# Autodesk Inventor assembly: Übung KO2 2023
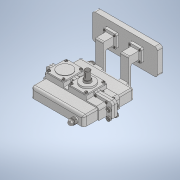
[picture p0: Inventor's stored thumbnail of the model, 180x180]
Saved by Autodesk Inventor 2022 (Build 260153000, 153)
## iProperties
Created: 2023-01-26
Part Number: Übung KO2 2023
Document SubType Name: Assembly
Designer: Matias Nicky
Author: Matias Nicky
## Documents named in this file (26)
- C:\Users\Matias Nicky\Documents\Nicky\HTW Fahrzeugtechnik\Semester 4\Konstruktion 2\Inventor\Übung KO2 2023.iam
- C:\Users\Matias Nicky\Documents\Nicky\HTW Fahrzeugtechnik\Semester 4\Konstruktion 2\Inventor\AbtriebswelleZahnrad 2.ipt
- C:\Users\Matias Nicky\Documents\Nicky\HTW Fahrzeugtechnik\Semester 4\Konstruktion 2\Inventor\AntriebswelleZahnrad 1.ipt
- C:\Users\Matias Nicky\Documents\Nicky\HTW Fahrzeugtechnik\Semester 4\Konstruktion 2\Inventor\Zahnrad2Rad2.ipt
- C:\Users\Matias Nicky\Documents\Inventor\Content Center Files\R2022\de-DE\DIN 471(2)\DIN 471 - 30 x 1,5(1).ipt
- C:\Users\Matias Nicky\Documents\Inventor\Content Center Files\R2022\de-DE\DIN 471(2)\DIN 471 - 35 x 1,5(1).ipt
- C:\Users\Matias Nicky\Documents\Inventor\Content Center Files\R2022\de-DE\DIN BEARING(1)\DIN 625 SKF - SKF 6006.ipt
- C:\Users\Matias Nicky\Documents\Nicky\HTW Fahrzeugtechnik\Semester 4\Konstruktion 2\Inventor\Gehäuse.ipt
- C:\Users\Matias Nicky\Documents\Nicky\HTW Fahrzeugtechnik\Semester 4\Konstruktion 2\Inventor\Gehäuse oben.ipt
- C:\Users\Matias Nicky\Documents\Inventor\Content Center Files\R2022\de-DE\DIN 3771(00)\DIN 3771 - 60 x 3,55 - N - NBR 70(1).ipt
- C:\Users\Matias Nicky\Documents\Inventor\Content Center Files\R2022\de-DE\DIN 6912\DIN 6912 - M10 x 30.ipt
- C:\Users\Matias Nicky\Documents\Inventor\Content Center Files\R2022\de-DE\ISO 4032(1)\ISO 4032 - M10DIN EN.ipt
- C:\Users\Matias Nicky\Documents\Inventor\Content Center Files\R2022\de-DE\DIN 6912\DIN 6912 - M6 x 30.ipt
- C:\Users\Matias Nicky\Documents\Inventor\Content Center Files\R2022\de-DE\DIN 6912\DIN 6912 - M5 x 30.ipt
- C:\Users\Matias Nicky\Documents\Inventor\Content Center Files\R2022\de-DE\ISO 4032(1)\ISO 4032 - M6DIN EN.ipt
- C:\Users\Matias Nicky\Documents\Inventor\Content Center Files\R2022\de-DE\ISO 4032(1)\ISO 4032 - M5DIN EN.ipt
- C:\Users\Matias Nicky\Documents\Nicky\HTW Fahrzeugtechnik\Semester 4\Konstruktion 2\Inventor\Deckel Endewelle.ipt
- C:\Users\Matias Nicky\Documents\Inventor\Content Center Files\R2022\de-DE\IS 7483\IS 7483 - M5 x 10.ipt
- C:\Users\Matias Nicky\Documents\Nicky\HTW Fahrzeugtechnik\Semester 4\Konstruktion 2\Inventor\Deckel verbindungswelle.ipt
- C:\Users\Matias Nicky\Documents\Inventor\Content Center Files\R2022\de-DE\ISO 6194_1(2)\ISO 6194_1 - 25x47x7-Typ 2.ipt
- C:\Users\Matias Nicky\Documents\Inventor\Content Center Files\R2022\de-DE\DIN 1587\DIN 1587 - M14 x 2.ipt
- C:\Users\Matias Nicky\Documents\Nicky\HTW Fahrzeugtechnik\Semester 4\Konstruktion 2\Inventor\Schmierung.ipt
- C:\Users\Matias Nicky\Documents\Inventor\Content Center Files\R2022\de-DE\DIN 6885-1 A\DIN 6885 - A 10 x 8 x 22.ipt
- C:\Users\Matias Nicky\Documents\Nicky\HTW Fahrzeugtechnik\Semester 4\Konstruktion 2\Inventor\Platte für Gehäuse.ipt
- C:\Users\Matias Nicky\Documents\Inventor\Content Center Files\R2022\de-DE\DIN 920\DIN 920 - M5 x 16.ipt
- C:\Users\Matias Nicky\Documents\Nicky\HTW Fahrzeugtechnik\Semester 4\Konstruktion 2\Inventor\Gehäuse festigung platte.ipt
## Components (94 placed, 25 different names)
1. AbtriebswelleZahnrad 2:1 — Passend:21, Passend:22, Passend:23, Passend:24, Passend:29, Passend:30, Passend:35, Fluchtend:1, Passend:38, Passend:40, Passend:47, Passend:98, Passend:102, Passend:126, Passend:129, Passend:133, Passend:134, Passend:135
2. AntriebswelleZahnrad 1:1 — Passend:17, Passend:25, Passend:26, Passend:27, Passend:28, Passend:35, Fluchtend:1, Passend:37, Passend:46, Passend:99, Passend:101, Passend:127, Passend:164
3. Zahnrad2Rad2:1 — Passend:126, Passend:129
4. DIN 471 > 9mm <= 300mm 30 x 1,5:2 — Passend:21, Passend:22, Passend:39
5. DIN 471 > 9mm <= 300mm 30 x 1,5:5 — Passend:23, Passend:24, Passend:43
6. DIN 471 > 9mm <= 300mm 35 x 1,5:1 — Passend:29, Passend:30
7. DIN 471 > 9mm <= 300mm 30 x 1,5:3 — Passend:17, Passend:25, Passend:26, Passend:44
8. DIN 471 > 9mm <= 300mm 30 x 1,5:4 — Passend:27, Passend:28, Passend:128
9. DIN 625 SKF SKF 6006:1 — Passend:19, Passend:38, Passend:43
10. DIN 625 SKF SKF 6006:2 — Passend:20, Passend:39, Passend:41, Passend:45
11. DIN 625 SKF SKF 6006:3 — Passend:32, Passend:37, Passend:42, Passend:127, Passend:128
12. DIN 625 SKF SKF 6006:4 — Passend:31, Passend:44
13. Gehäuse:1 — Passend:18, Passend:19, Passend:20, Passend:31, Passend:32, Passend:41, Passend:42, Passend:61, Passend:63, Passend:65, Passend:67, Passend:73, Passend:75, Passend:77, Passend:79, Passend:81, Passend:83, Einfügen:17, Einfügen:18, Passend:84, Fluchtend:6, Passend:85, Passend:86, Fluchtend:7, Passend:87, Passend:96, Passend:97, Passend:100, Passend:103, Passend:104, Passend:105, Passend:124, Passend:125, Fluchtend:8, Passend:130, Passend:131, Passend:132, Passend:136, Passend:137, Passend:138, Passend:139, Passend:140, Passend:141
14. Gehäuse oben:1 — Passend:18, Passend:40, Passend:45, Fluchtend:3, Fluchtend:5, Passend:50, Passend:51, Passend:52, Passend:53, Passend:56, Passend:57, Passend:58, Passend:59, Einfügen:9, Einfügen:10, Einfügen:11, Einfügen:12, Einfügen:13, Einfügen:14, Einfügen:15, Einfügen:16, Passend:122, Passend:123
15. DIN 3771 60 x 3,55 - N - NBR 70:1 — Passend:47, Fluchtend:2
16. DIN 3771 60 x 3,55 - N - NBR 70:2 — Passend:46, Fluchtend:4
17. DIN 6912 M10 x 30:5 — Passend:50, Passend:51, Passend:66
18. DIN 6912 M10 x 30:3 — Passend:52, Passend:53, Passend:60
19. DIN 6912 M10 x 30:2 — Passend:56, Passend:57, Passend:62
20. DIN 6912 M10 x 30:6 — Passend:58, Passend:59, Passend:64
21. DIN EN 24032 M10:1 — Passend:60, Passend:61
22. DIN EN 24032 M10:2 — Passend:62, Passend:63
23. DIN EN 24032 M10:3 — Passend:64, Passend:65
24. DIN EN 24032 M10:4 — Passend:66, Passend:67
25. DIN 6912 M5 x 30:1 — Einfügen:9, Passend:82
26. DIN 6912 M5 x 30:2 — Einfügen:10, Passend:80
27. DIN 6912 M5 x 30:3 — Einfügen:11, Passend:76
28. DIN 6912 M5 x 30:4 — Einfügen:12, Passend:72
29. DIN 6912 M5 x 30:5 — Einfügen:13, Passend:74
30. DIN 6912 M5 x 30:6 — Einfügen:14, Passend:78
31. DIN EN 24032 M5:1 — Passend:72, Passend:73
32. DIN EN 24032 M5:2 — Passend:74, Passend:75
33. DIN EN 24032 M5:3 — Passend:76, Passend:77
34. DIN EN 24032 M5:4 — Passend:78, Passend:79
35. DIN EN 24032 M5:5 — Passend:80, Passend:81
36. DIN EN 24032 M5:6 — Passend:82, Passend:83
37. DIN 6912 M6 x 30:1 — Einfügen:15
38. DIN 6912 M6 x 30:2 — Einfügen:16
39. DIN EN 24032 M6:1 — Einfügen:17
40. DIN EN 24032 M6:2 — Einfügen:18
41. Deckel Endewelle:1 — Passend:84, Fluchtend:6, Passend:85, Passend:88, Passend:89, Passend:90, Passend:91, Passend:92, Passend:93, Passend:94, Passend:95
42. Deckel Endewelle:2 — Passend:86, Fluchtend:7, Passend:87, Einfügen:19, Einfügen:20, Einfügen:21, Einfügen:22
43. IS 7483 M5 x 10:1 — Passend:88, Passend:89
44. IS 7483 M5 x 10:2 — Passend:90, Passend:91
45. IS 7483 M5 x 10:3 — Passend:92, Passend:93
46. IS 7483 M5 x 10:4 — Passend:94, Passend:95
47. IS 7483 M5 x 10:5 — Einfügen:19
48. IS 7483 M5 x 10:6 — Einfügen:20
49. IS 7483 M5 x 10:7 — Einfügen:21
50. IS 7483 M5 x 10:8 — Einfügen:22
51. Deckel verbindungswelle:1 — Passend:96, Passend:97, Passend:103, Passend:114, Passend:115, Passend:116, Passend:117, Passend:118, Passend:119, Passend:120, Passend:121
52. Deckel verbindungswelle:2 — Passend:100, Passend:104, Passend:105, Passend:106, Passend:107, Passend:108, Passend:109, Passend:110, Passend:111, Passend:112, Passend:113
53. ISO 6194/1 25x47x7-Typ 2:1 — Passend:98, Passend:102
54. ISO 6194/1 25x47x7-Typ 2:2 — Passend:99, Passend:101
55. IS 7483 M5 x 10:9 — Passend:106, Passend:107
56. IS 7483 M5 x 10:10 — Passend:108, Passend:109
57. IS 7483 M5 x 10:11 — Passend:110, Passend:111
58. IS 7483 M5 x 10:12 — Passend:112, Passend:113
59. IS 7483 M5 x 10:13 — Passend:114, Passend:115
60. IS 7483 M5 x 10:14 — Passend:116, Passend:117
61. IS 7483 M5 x 10:15 — Passend:118, Passend:119
62. IS 7483 M5 x 10:16 — Passend:120, Passend:121
63. DIN 1587 M14 - SW21:1 — Passend:122, Passend:123
64. DIN 1587 M14 - SW21:2 — Passend:124, Passend:125
65. Schmierung:1 — Passend:130, Passend:131, Passend:132
66. DIN 6885-1 A A 10 x 8 x 22:1 — Passend:133, Passend:134, Passend:135
67. Platte für Gehäuse:1 — Passend:139, Passend:140, Passend:141, Einfügen:23, Einfügen:24, Einfügen:25, Einfügen:26, Passend:142, Passend:143, Passend:144, Passend:146, Passend:148, Passend:149, Passend:150, Passend:151, Passend:152, Passend:153, Passend:154, Passend:155, Passend:156, Passend:157, Passend:158, Passend:159, Passend:160, Passend:161, Passend:162, Passend:163
68. Platte für Gehäuse:2 — Passend:136, Passend:137, Passend:138, Einfügen:27, Einfügen:28, Einfügen:29, Einfügen:30, Passend:145, Passend:147, Einfügen:31, Einfügen:32, Einfügen:33, Einfügen:34, Einfügen:35, Einfügen:36, Einfügen:37, Einfügen:38
69. DIN 920 M5 x 16:1 — Einfügen:23
70. DIN 920 M5 x 16:2 — Einfügen:24
71. DIN 920 M5 x 16:3 — Einfügen:25
72. DIN 920 M5 x 16:4 — Einfügen:26
73. DIN 920 M5 x 16:5 — Einfügen:27
74. DIN 920 M5 x 16:6 — Einfügen:28
75. DIN 920 M5 x 16:7 — Einfügen:29
76. DIN 920 M5 x 16:8 — Einfügen:30
77. Gehäuse festigung platte:1 — Passend:142, Passend:143, Passend:144
78. Gehäuse festigung platte:2 — Passend:145, Passend:146, Passend:147
79. DIN 920 M5 x 16:9 — Passend:148, Passend:149
80. DIN 920 M5 x 16:10 — Passend:150, Passend:151
81. DIN 920 M5 x 16:11 — Passend:152, Passend:153
82. DIN 920 M5 x 16:12 — Passend:154, Passend:155
83. DIN 920 M5 x 16:13 — Passend:156, Passend:157
84. DIN 920 M5 x 16:14 — Passend:158, Passend:159
85. DIN 920 M5 x 16:15 — Passend:160, Passend:161
86. DIN 920 M5 x 16:16 — Passend:162, Passend:163
87. DIN 920 M5 x 16:17 — Einfügen:31
88. DIN 920 M5 x 16:18 — Einfügen:32
89. DIN 920 M5 x 16:19 — Einfügen:33
90. DIN 920 M5 x 16:20 — Einfügen:34
91. DIN 920 M5 x 16:21 — Einfügen:35
92. DIN 920 M5 x 16:22 — Einfügen:36
93. DIN 920 M5 x 16:23 — Einfügen:37
94. DIN 920 M5 x 16:24 — Einfügen:38
## Relationships (175: Mate 137, Insert 30, Flush 8)
- Passend:17 [Mate]: AntriebswelleZahnrad 1:1 ↔ DIN 471 > 9mm <= 300mm 30 x 1,5:3
- Passend:18 [Mate]: Gehäuse:1 ↔ Gehäuse oben:1
- Passend:19 [Mate]: DIN 625 SKF SKF 6006:1 ↔ Gehäuse:1
- Passend:20 [Mate]: DIN 625 SKF SKF 6006:2 ↔ Gehäuse:1
- Passend:21 [Mate]: AbtriebswelleZahnrad 2:1 ↔ DIN 471 > 9mm <= 300mm 30 x 1,5:2
- Passend:22 [Mate]: AbtriebswelleZahnrad 2:1 ↔ DIN 471 > 9mm <= 300mm 30 x 1,5:2
- Passend:23 [Mate]: AbtriebswelleZahnrad 2:1 ↔ DIN 471 > 9mm <= 300mm 30 x 1,5:5
- Passend:24 [Mate]: AbtriebswelleZahnrad 2:1 ↔ DIN 471 > 9mm <= 300mm 30 x 1,5:5
- Passend:25 [Mate]: AntriebswelleZahnrad 1:1 ↔ DIN 471 > 9mm <= 300mm 30 x 1,5:3
- Passend:26 [Mate]: AntriebswelleZahnrad 1:1 ↔ DIN 471 > 9mm <= 300mm 30 x 1,5:3
- Passend:27 [Mate]: AntriebswelleZahnrad 1:1 ↔ DIN 471 > 9mm <= 300mm 30 x 1,5:4
- Passend:28 [Mate]: AntriebswelleZahnrad 1:1 ↔ DIN 471 > 9mm <= 300mm 30 x 1,5:4
- Passend:29 [Mate]: AbtriebswelleZahnrad 2:1 ↔ DIN 471 > 9mm <= 300mm 35 x 1,5:1
- Passend:30 [Mate]: AbtriebswelleZahnrad 2:1 ↔ DIN 471 > 9mm <= 300mm 35 x 1,5:1
- Passend:31 [Mate]: DIN 625 SKF SKF 6006:4 ↔ Gehäuse:1
- Passend:32 [Mate]: DIN 625 SKF SKF 6006:3 ↔ Gehäuse:1
- Passend:35 [Mate] (87 mm): AbtriebswelleZahnrad 2:1 ↔ AntriebswelleZahnrad 1:1
- Fluchtend:1 [Flush]: AbtriebswelleZahnrad 2:1 ↔ AntriebswelleZahnrad 1:1
- Passend:37 [Mate]: AntriebswelleZahnrad 1:1 ↔ DIN 625 SKF SKF 6006:3
- Passend:38 [Mate]: AbtriebswelleZahnrad 2:1 ↔ DIN 625 SKF SKF 6006:1
- Passend:39 [Mate]: DIN 471 > 9mm <= 300mm 30 x 1,5:2 ↔ DIN 625 SKF SKF 6006:2
- Passend:40 [Mate]: AbtriebswelleZahnrad 2:1 ↔ Gehäuse oben:1
- Passend:41 [Mate]: DIN 625 SKF SKF 6006:2 ↔ Gehäuse:1
- Passend:42 [Mate]: DIN 625 SKF SKF 6006:3 ↔ Gehäuse:1
- Passend:43 [Mate]: DIN 471 > 9mm <= 300mm 30 x 1,5:5 ↔ DIN 625 SKF SKF 6006:1
- Passend:44 [Mate]: DIN 471 > 9mm <= 300mm 30 x 1,5:3 ↔ DIN 625 SKF SKF 6006:4
- Passend:45 [Mate]: DIN 625 SKF SKF 6006:2 ↔ Gehäuse oben:1
- Passend:46 [Mate]: AntriebswelleZahnrad 1:1 ↔ DIN 3771 60 x 3,55 - N - NBR 70:2
- Passend:47 [Mate]: AbtriebswelleZahnrad 2:1 ↔ DIN 3771 60 x 3,55 - N - NBR 70:1
- Fluchtend:2 [Flush] (-1.775 mm): DIN 3771 60 x 3,55 - N - NBR 70:1
- Fluchtend:3 [Flush]: Gehäuse oben:1
- Fluchtend:4 [Flush] (-1.755 mm): DIN 3771 60 x 3,55 - N - NBR 70:2
- Fluchtend:5 [Flush]: Gehäuse oben:1
- Passend:50 [Mate]: Gehäuse oben:1 ↔ DIN 6912 M10 x 30:5
- Passend:51 [Mate]: Gehäuse oben:1 ↔ DIN 6912 M10 x 30:5
- Passend:52 [Mate]: Gehäuse oben:1 ↔ DIN 6912 M10 x 30:3
- Passend:53 [Mate]: Gehäuse oben:1 ↔ DIN 6912 M10 x 30:3
- Passend:56 [Mate]: Gehäuse oben:1 ↔ DIN 6912 M10 x 30:2
- Passend:57 [Mate]: Gehäuse oben:1 ↔ DIN 6912 M10 x 30:2
- Passend:58 [Mate]: Gehäuse oben:1 ↔ DIN 6912 M10 x 30:6
- Passend:59 [Mate]: Gehäuse oben:1 ↔ DIN 6912 M10 x 30:6
- Passend:60 [Mate]: DIN 6912 M10 x 30:3 ↔ DIN EN 24032 M10:1
- Passend:61 [Mate]: Gehäuse:1 ↔ DIN EN 24032 M10:1
- Passend:62 [Mate]: DIN 6912 M10 x 30:2 ↔ DIN EN 24032 M10:2
- Passend:63 [Mate]: Gehäuse:1 ↔ DIN EN 24032 M10:2
- Passend:64 [Mate]: DIN 6912 M10 x 30:6 ↔ DIN EN 24032 M10:3
- Passend:65 [Mate]: Gehäuse:1 ↔ DIN EN 24032 M10:3
- Passend:66 [Mate]: DIN 6912 M10 x 30:5 ↔ DIN EN 24032 M10:4
- Passend:67 [Mate]: Gehäuse:1 ↔ DIN EN 24032 M10:4
- Einfügen:9 [Insert]: Gehäuse oben:1 ↔ DIN 6912 M5 x 30:1
- Einfügen:10 [Insert]: Gehäuse oben:1 ↔ DIN 6912 M5 x 30:2
- Einfügen:11 [Insert]: Gehäuse oben:1 ↔ DIN 6912 M5 x 30:3
- Einfügen:12 [Insert]: Gehäuse oben:1 ↔ DIN 6912 M5 x 30:4
- Einfügen:13 [Insert]: Gehäuse oben:1 ↔ DIN 6912 M5 x 30:5
- Einfügen:14 [Insert]: Gehäuse oben:1 ↔ DIN 6912 M5 x 30:6
- Passend:72 [Mate]: DIN 6912 M5 x 30:4 ↔ DIN EN 24032 M5:1
- Passend:73 [Mate]: Gehäuse:1 ↔ DIN EN 24032 M5:1
- Passend:74 [Mate]: DIN 6912 M5 x 30:5 ↔ DIN EN 24032 M5:2
- Passend:75 [Mate]: Gehäuse:1 ↔ DIN EN 24032 M5:2
- Passend:76 [Mate]: DIN 6912 M5 x 30:3 ↔ DIN EN 24032 M5:3
- Passend:77 [Mate]: Gehäuse:1 ↔ DIN EN 24032 M5:3
- Passend:78 [Mate]: DIN 6912 M5 x 30:6 ↔ DIN EN 24032 M5:4
- Passend:79 [Mate]: Gehäuse:1 ↔ DIN EN 24032 M5:4
- Passend:80 [Mate]: DIN 6912 M5 x 30:2 ↔ DIN EN 24032 M5:5
- Passend:81 [Mate]: Gehäuse:1 ↔ DIN EN 24032 M5:5
- Passend:82 [Mate]: DIN 6912 M5 x 30:1 ↔ DIN EN 24032 M5:6
- Passend:83 [Mate]: Gehäuse:1 ↔ DIN EN 24032 M5:6
- Einfügen:15 [Insert]: Gehäuse oben:1 ↔ DIN 6912 M6 x 30:1
- Einfügen:16 [Insert]: Gehäuse oben:1 ↔ DIN 6912 M6 x 30:2
- Einfügen:17 [Insert]: Gehäuse:1 ↔ DIN EN 24032 M6:1
- Einfügen:18 [Insert]: Gehäuse:1 ↔ DIN EN 24032 M6:2
- Passend:84 [Mate]: Gehäuse:1 ↔ Deckel Endewelle:1
- Fluchtend:6 [Flush]: Gehäuse:1 ↔ Deckel Endewelle:1
- Passend:85 [Mate]: Gehäuse:1 ↔ Deckel Endewelle:1
- Passend:86 [Mate]: Gehäuse:1 ↔ Deckel Endewelle:2
- Fluchtend:7 [Flush]: Gehäuse:1 ↔ Deckel Endewelle:2
- Passend:87 [Mate]: Gehäuse:1 ↔ Deckel Endewelle:2
- Passend:88 [Mate]: Deckel Endewelle:1 ↔ IS 7483 M5 x 10:1
- Passend:89 [Mate]: Deckel Endewelle:1 ↔ IS 7483 M5 x 10:1
- Passend:90 [Mate]: Deckel Endewelle:1 ↔ IS 7483 M5 x 10:2
- Passend:91 [Mate]: Deckel Endewelle:1 ↔ IS 7483 M5 x 10:2
- Passend:92 [Mate]: Deckel Endewelle:1 ↔ IS 7483 M5 x 10:3
- Passend:93 [Mate]: Deckel Endewelle:1 ↔ IS 7483 M5 x 10:3
- Passend:94 [Mate]: Deckel Endewelle:1 ↔ IS 7483 M5 x 10:4
- Passend:95 [Mate]: Deckel Endewelle:1 ↔ IS 7483 M5 x 10:4
- Einfügen:19 [Insert]: Deckel Endewelle:2 ↔ IS 7483 M5 x 10:5
- Einfügen:20 [Insert]: Deckel Endewelle:2 ↔ IS 7483 M5 x 10:6
- Einfügen:21 [Insert]: Deckel Endewelle:2 ↔ IS 7483 M5 x 10:7
- Einfügen:22 [Insert]: Deckel Endewelle:2 ↔ IS 7483 M5 x 10:8
- Passend:96 [Mate]: Gehäuse:1 ↔ Deckel verbindungswelle:1
- Passend:97 [Mate]: Gehäuse:1 ↔ Deckel verbindungswelle:1
- Passend:98 [Mate]: AbtriebswelleZahnrad 2:1 ↔ ISO 6194/1 25x47x7-Typ 2:1
- Passend:99 [Mate]: AntriebswelleZahnrad 1:1 ↔ ISO 6194/1 25x47x7-Typ 2:2
- Passend:100 [Mate]: Gehäuse:1 ↔ Deckel verbindungswelle:2
- Passend:101 [Mate]: AntriebswelleZahnrad 1:1 ↔ ISO 6194/1 25x47x7-Typ 2:2
- Passend:102 [Mate]: AbtriebswelleZahnrad 2:1 ↔ ISO 6194/1 25x47x7-Typ 2:1
- Passend:103 [Mate]: Gehäuse:1 ↔ Deckel verbindungswelle:1
- Passend:104 [Mate]: Gehäuse:1 ↔ Deckel verbindungswelle:2
- Passend:105 [Mate]: Gehäuse:1 ↔ Deckel verbindungswelle:2
- Passend:106 [Mate]: Deckel verbindungswelle:2 ↔ IS 7483 M5 x 10:9
- Passend:107 [Mate]: Deckel verbindungswelle:2 ↔ IS 7483 M5 x 10:9
- Passend:108 [Mate]: Deckel verbindungswelle:2 ↔ IS 7483 M5 x 10:10
- Passend:109 [Mate]: Deckel verbindungswelle:2 ↔ IS 7483 M5 x 10:10
- Passend:110 [Mate]: Deckel verbindungswelle:2 ↔ IS 7483 M5 x 10:11
- Passend:111 [Mate]: Deckel verbindungswelle:2 ↔ IS 7483 M5 x 10:11
- Passend:112 [Mate]: Deckel verbindungswelle:2 ↔ IS 7483 M5 x 10:12
- Passend:113 [Mate]: Deckel verbindungswelle:2 ↔ IS 7483 M5 x 10:12
- Passend:114 [Mate]: Deckel verbindungswelle:1 ↔ IS 7483 M5 x 10:13
- Passend:115 [Mate]: Deckel verbindungswelle:1 ↔ IS 7483 M5 x 10:13
- Passend:116 [Mate]: Deckel verbindungswelle:1 ↔ IS 7483 M5 x 10:14
- Passend:117 [Mate]: Deckel verbindungswelle:1 ↔ IS 7483 M5 x 10:14
- Passend:118 [Mate]: Deckel verbindungswelle:1 ↔ IS 7483 M5 x 10:15
- Passend:119 [Mate]: Deckel verbindungswelle:1 ↔ IS 7483 M5 x 10:15
- Passend:120 [Mate]: Deckel verbindungswelle:1 ↔ IS 7483 M5 x 10:16
- Passend:121 [Mate]: Deckel verbindungswelle:1 ↔ IS 7483 M5 x 10:16
- Passend:122 [Mate]: Gehäuse oben:1 ↔ DIN 1587 M14 - SW21:1
- Passend:123 [Mate]: Gehäuse oben:1 ↔ DIN 1587 M14 - SW21:1
- Passend:124 [Mate]: Gehäuse:1 ↔ DIN 1587 M14 - SW21:2
- Passend:125 [Mate]: Gehäuse:1 ↔ DIN 1587 M14 - SW21:2
- Passend:126 [Mate]: AbtriebswelleZahnrad 2:1 ↔ Zahnrad2Rad2:1
- Passend:127 [Mate]: AntriebswelleZahnrad 1:1 ↔ DIN 625 SKF SKF 6006:3
- Passend:128 [Mate]: DIN 471 > 9mm <= 300mm 30 x 1,5:4 ↔ DIN 625 SKF SKF 6006:3
- Passend:129 [Mate]: AbtriebswelleZahnrad 2:1 ↔ Zahnrad2Rad2:1
- Fluchtend:8 [Flush]: Gehäuse:1
- Passend:130 [Mate]: Gehäuse:1 ↔ Schmierung:1
- Passend:131 [Mate]: Gehäuse:1 ↔ Schmierung:1
- Passend:132 [Mate]: Gehäuse:1 ↔ Schmierung:1
- Passend:133 [Mate]: AbtriebswelleZahnrad 2:1 ↔ DIN 6885-1 A A 10 x 8 x 22:1
- Passend:134 [Mate]: AbtriebswelleZahnrad 2:1 ↔ DIN 6885-1 A A 10 x 8 x 22:1
- Passend:135 [Mate]: AbtriebswelleZahnrad 2:1 ↔ DIN 6885-1 A A 10 x 8 x 22:1
- Passend:136 [Mate]: Gehäuse:1 ↔ Platte für Gehäuse:2
- Passend:137 [Mate]: Gehäuse:1 ↔ Platte für Gehäuse:2
- Passend:138 [Mate]: Gehäuse:1 ↔ Platte für Gehäuse:2
- Passend:139 [Mate]: Gehäuse:1 ↔ Platte für Gehäuse:1
- Passend:140 [Mate]: Gehäuse:1 ↔ Platte für Gehäuse:1
- Passend:141 [Mate]: Gehäuse:1 ↔ Platte für Gehäuse:1
- Einfügen:23 [Insert]: Platte für Gehäuse:1 ↔ DIN 920 M5 x 16:1
- Einfügen:24 [Insert]: Platte für Gehäuse:1 ↔ DIN 920 M5 x 16:2
- Einfügen:25 [Insert]: Platte für Gehäuse:1 ↔ DIN 920 M5 x 16:3
- Einfügen:26 [Insert]: Platte für Gehäuse:1 ↔ DIN 920 M5 x 16:4
- Einfügen:27 [Insert]: Platte für Gehäuse:2 ↔ DIN 920 M5 x 16:5
- Einfügen:28 [Insert]: Platte für Gehäuse:2 ↔ DIN 920 M5 x 16:6
- Einfügen:29 [Insert]: Platte für Gehäuse:2 ↔ DIN 920 M5 x 16:7
- Einfügen:30 [Insert]: Platte für Gehäuse:2 ↔ DIN 920 M5 x 16:8
- Passend:142 [Mate]: Platte für Gehäuse:1 ↔ Gehäuse festigung platte:1
- Passend:143 [Mate]: Platte für Gehäuse:1 ↔ Gehäuse festigung platte:1
- Passend:144 [Mate]: Platte für Gehäuse:1 ↔ Gehäuse festigung platte:1
- Passend:145 [Mate]: Platte für Gehäuse:2 ↔ Gehäuse festigung platte:2
- Passend:146 [Mate]: Platte für Gehäuse:1 ↔ Gehäuse festigung platte:2
- Passend:147 [Mate]: Platte für Gehäuse:2 ↔ Gehäuse festigung platte:2
- Passend:148 [Mate]: Platte für Gehäuse:1 ↔ DIN 920 M5 x 16:9
- Passend:149 [Mate]: Platte für Gehäuse:1 ↔ DIN 920 M5 x 16:9
- Passend:150 [Mate]: Platte für Gehäuse:1 ↔ DIN 920 M5 x 16:10
- Passend:151 [Mate]: Platte für Gehäuse:1 ↔ DIN 920 M5 x 16:10
- Passend:152 [Mate]: Platte für Gehäuse:1 ↔ DIN 920 M5 x 16:11
- Passend:153 [Mate]: Platte für Gehäuse:1 ↔ DIN 920 M5 x 16:11
- Passend:154 [Mate]: Platte für Gehäuse:1 ↔ DIN 920 M5 x 16:12
- Passend:155 [Mate]: Platte für Gehäuse:1 ↔ DIN 920 M5 x 16:12
- Passend:156 [Mate]: Platte für Gehäuse:1 ↔ DIN 920 M5 x 16:13
- Passend:157 [Mate]: Platte für Gehäuse:1 ↔ DIN 920 M5 x 16:13
- Passend:158 [Mate]: Platte für Gehäuse:1 ↔ DIN 920 M5 x 16:14
- Passend:159 [Mate]: Platte für Gehäuse:1 ↔ DIN 920 M5 x 16:14
- Passend:160 [Mate]: Platte für Gehäuse:1 ↔ DIN 920 M5 x 16:15
- Passend:161 [Mate]: Platte für Gehäuse:1 ↔ DIN 920 M5 x 16:15
- Passend:162 [Mate]: Platte für Gehäuse:1 ↔ DIN 920 M5 x 16:16
- Passend:163 [Mate]: Platte für Gehäuse:1 ↔ DIN 920 M5 x 16:16
- Einfügen:31 [Insert]: Platte für Gehäuse:2 ↔ DIN 920 M5 x 16:17
- Einfügen:32 [Insert]: Platte für Gehäuse:2 ↔ DIN 920 M5 x 16:18
- Einfügen:33 [Insert]: Platte für Gehäuse:2 ↔ DIN 920 M5 x 16:19
- Einfügen:34 [Insert]: Platte für Gehäuse:2 ↔ DIN 920 M5 x 16:20
- Einfügen:35 [Insert]: Platte für Gehäuse:2 ↔ DIN 920 M5 x 16:21
- Einfügen:36 [Insert]: Platte für Gehäuse:2 ↔ DIN 920 M5 x 16:22
- Einfügen:37 [Insert]: Platte für Gehäuse:2 ↔ DIN 920 M5 x 16:23
- Einfügen:38 [Insert]: Platte für Gehäuse:2 ↔ DIN 920 M5 x 16:24
- Passend:164 [Mate]: AntriebswelleZahnrad 1:1
